# Autodesk Inventor assembly: ASY сальниковый узел
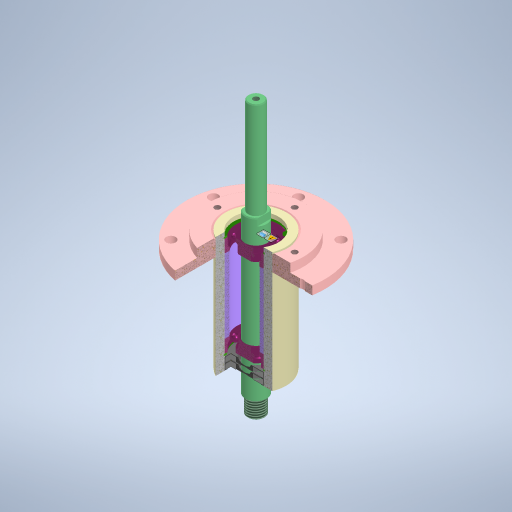
[picture p0: Inventor's stored thumbnail of the model, 512x512]
Saved by Autodesk Inventor 2024.2 (Build 282272000, 272)
## iProperties
Created: 2024-03-01
Part Number: ASY сальниковый узел
Document SubType Name: Assembly
Designer: admin
Author: admin
## Documents named in this file (8)
- C:\Users\pokla\Documents\Inventor\Мешалка\хвосты\ASY сальниковый узел.iam
- C:\Users\pokla\Documents\Inventor\Мешалка\хвосты\Втулка 1.ipt
- C:\Users\pokla\Documents\Inventor\Мешалка\хвосты\Блин.ipt
- C:\Users\pokla\Documents\Inventor\Мешалка\хвосты\Вал.ipt
- C:\Users\pokla\Documents\Inventor\Мешалка\хвосты\SKF B7205 BE.ipt
- C:\Users\pokla\Documents\Inventor\Мешалка\хвосты\ISO 6194_1 - 25x52x7-Type 3.ipt
- C:\Users\pokla\Documents\Inventor\Мешалка\хвосты\ANSI B 27.7M - 3BMI-52.ipt
- C:\Users\pokla\Documents\Inventor\Мешалка\хвосты\дистанс.втулка.ipt
## Components (10 placed, 7 different names)
1. Втулка 1:1 — Mate:2, Flush:1
2. Блин:1 — Mate:1
3. ANSI B 27.7M 3BMI-52:1
4. SKF B- Angular contact SKF B7205 BE:1 — Rotational:8
5. дистанс.втулка:1 — Rotational:8
6. SKF B- Angular contact SKF B7205 BE:2
7. ANSI B 27.7M 3BMI-52:2
8. ISO 6194/1 25x52x7-Type 3:2
9. ISO 6194/1 25x52x7-Type 3:1
10. Вал:1
## Relationships (11: RevoluteJoint 7, Mate 2, WeldJoint 1, Flush 1)
- [WeldJoint]: Втулка 1:1 ↔ Блин:1
- [RevoluteJoint]: Втулка 1:1 ↔ SKF B- Angular contact SKF B7205 BE:1
- [RevoluteJoint]: Втулка 1:1 ↔ SKF B- Angular contact SKF B7205 BE:2
- [RevoluteJoint]: Втулка 1:1 ↔ ANSI B 27.7M 3BMI-52:1
- [RevoluteJoint]: Втулка 1:1 ↔ ISO 6194/1 25x52x7-Type 3:1
- [RevoluteJoint]: ISO 6194/1 25x52x7-Type 3:2 ↔ ISO 6194/1 25x52x7-Type 3:1
- [RevoluteJoint]: Втулка 1:1 ↔ ANSI B 27.7M 3BMI-52:2
- Mate:1: Блин:1
- Mate:2: Втулка 1:1
- Flush:1: Втулка 1:1
- Rotational:8 [RevoluteJoint]: SKF B- Angular contact SKF B7205 BE:1 ↔ дистанс.втулка:1
